# Autodesk Inventor assembly: SE Matriz Centelladora DC
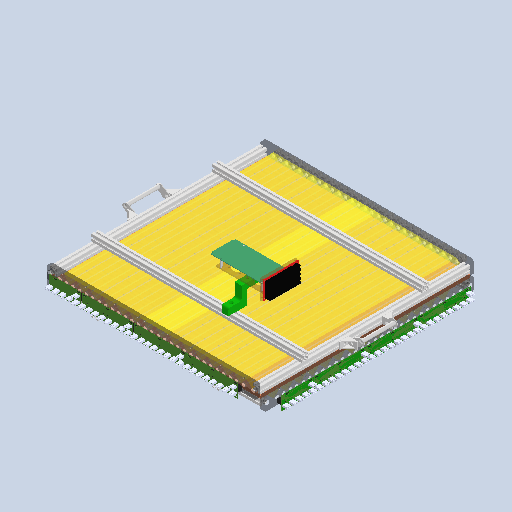
[picture p0: Inventor's stored thumbnail of the model, 512x512]
Saved by Autodesk Inventor 2024.2 (Build 282272000, 272)
## iProperties
Created: 2025-11-07
Part Number: SE Matriz Centelladora DC
Document SubType Name: Assembly
Designer: ja.restrepo1
Author: ja.restrepo1
## Documents named in this file (8)
- I:\MICROMECANICA\ALTAS ENERGIAS\Deteccion de Muones\Detectores centelladores\Partes Detector Centellador\SE Matriz Centelladora DC\SE Matriz Centelladora DC.iam
- I:\MICROMECANICA\ALTAS ENERGIAS\Deteccion de Muones\Detectores centelladores\Partes Detector Centellador\SE Matriz Centelladora DC\Soporte de matriz centelladora.ipt
- I:\MICROMECANICA\ALTAS ENERGIAS\Deteccion de Muones\Detectores centelladores\Partes Detector Centellador\SE Matriz Centelladora DC\SSE Matriz Centelladora 15X14\SSE Matriz centelladora 15X14.iam
- I:\MICROMECANICA\ALTAS ENERGIAS\Deteccion de Muones\Detectores centelladores\Partes Detector Centellador\SE Matriz Centelladora DC\SSE Estructura Centelladoras 20x20 DC\SSE estructura matriz centelladora.iam
- I:\MICROMECANICA\ALTAS ENERGIAS\Deteccion de Muones\Detectores centelladores\Partes Detector Centellador\SE Matriz Centelladora DC\SSE Manija\SSE. Manija.iam
- I:\MICROMECANICA\ALTAS ENERGIAS\Deteccion de Muones\Detectores centelladores\Partes Detector Centellador\SE Tarjetas IC DC\SSE tarjedas de AD DC.iam
- I:\MICROMECANICA\ALTAS ENERGIAS\Deteccion de Muones\Detectores centelladores\Partes Detector Centellador\SE Tarjetas IC DC\SSE SiPM 8CH Org.iam
- I:\MICROMECANICA\ALTAS ENERGIAS\Deteccion de Muones\Detectores centelladores\Partes Detector Centellador\SE Tarjetas IC DC\SSE SiPM 8Ch_2026.iam
## Components (10 placed, 7 different names)
1. Soporte de matriz centelladora:1 — Nivelación:1, Nivelación:2, Nivelación:3, Coincidencia:1, Coincidencia:2, Nivelación:4, Nivelación:5, Coincidencia:3, Nivelación:6, Nivelación:7, Coincidencia:4, Nivelación:8, Nivelación:9, Nivelación:10, Nivelación:11
2. SSE Matriz centelladora 15X14:1 [sub-assembly] — Coincidencia:2, Nivelación:4, Nivelación:6, Nivelación:7
3. SSE Matriz centelladora 15X14:2 [sub-assembly] — Nivelación:5, Coincidencia:3, Coincidencia:4
4. SSE estructura matriz centelladora:1 [sub-assembly] — Nivelación:8, Nivelación:9, Nivelación:10, Coincidencia:5, Nivelación:12, Coincidencia:6, Nivelación:13, Coincidencia:7, Ángulo:1, Nivelación:15, Coincidencia:8, Ángulo:2, Coincidencia:9, Nivelación:16, Coincidencia:10, Coincidencia:11, Nivelación:17, Nivelación:18, Coincidencia:12, Coincidencia:13
5. SSE. Manija:1 [sub-assembly] — Coincidencia:5, Nivelación:11, Nivelación:12, Nivelación:14
6. SSE. Manija:2 [sub-assembly] — Coincidencia:6, Nivelación:13, Nivelación:14
7. SSE tarjedas de AD DC:1 [sub-assembly] — Coincidencia:7, Ángulo:1, Nivelación:15
8. SSE SiPM 8CH Org:1 [sub-assembly] — Coincidencia:10, Coincidencia:11, Nivelación:17
9. SSE SiPM 8CH Org:2 [sub-assembly] — Coincidencia:8, Ángulo:2, Coincidencia:9, Nivelación:16
10. SSE SiPM 8Ch_2026:1 [sub-assembly] — Nivelación:18, Coincidencia:12, Coincidencia:13
## Relationships (33: Flush 18, Mate 13, Angle 2)
- Nivelación:1 [Flush]: Soporte de matriz centelladora:1
- Nivelación:2 [Flush]: Soporte de matriz centelladora:1
- Nivelación:3 [Flush]: Soporte de matriz centelladora:1
- Coincidencia:1 [Mate]: Soporte de matriz centelladora:1
- Coincidencia:2 [Mate]: Soporte de matriz centelladora:1 ↔ SSE Matriz centelladora 15X14:1
- Nivelación:4 [Flush]: Soporte de matriz centelladora:1 ↔ SSE Matriz centelladora 15X14:1
- Nivelación:5 [Flush]: Soporte de matriz centelladora:1 ↔ SSE Matriz centelladora 15X14:2
- Coincidencia:3 [Mate]: Soporte de matriz centelladora:1 ↔ SSE Matriz centelladora 15X14:2
- Nivelación:6 [Flush]: Soporte de matriz centelladora:1 ↔ SSE Matriz centelladora 15X14:1
- Nivelación:7 [Flush]: Soporte de matriz centelladora:1 ↔ SSE Matriz centelladora 15X14:1
- Coincidencia:4 [Mate]: Soporte de matriz centelladora:1 ↔ SSE Matriz centelladora 15X14:2
- Nivelación:8 [Flush]: Soporte de matriz centelladora:1 ↔ SSE estructura matriz centelladora:1
- Nivelación:9 [Flush]: Soporte de matriz centelladora:1 ↔ SSE estructura matriz centelladora:1
- Nivelación:10 [Flush]: Soporte de matriz centelladora:1 ↔ SSE estructura matriz centelladora:1
- Coincidencia:5 [Mate]: SSE estructura matriz centelladora:1 ↔ SSE. Manija:1
- Nivelación:11 [Flush]: Soporte de matriz centelladora:1 ↔ SSE. Manija:1
- Nivelación:12 [Flush] (0.5 mm): SSE estructura matriz centelladora:1 ↔ SSE. Manija:1
- Coincidencia:6 [Mate]: SSE estructura matriz centelladora:1 ↔ SSE. Manija:2
- Nivelación:13 [Flush] (-0.5 mm): SSE estructura matriz centelladora:1 ↔ SSE. Manija:2
- Nivelación:14 [Flush]: SSE. Manija:1 ↔ SSE. Manija:2
- Coincidencia:7 [Mate]: SSE estructura matriz centelladora:1 ↔ SSE tarjedas de AD DC:1
- Ángulo:1 [Angle] (0 deg): SSE estructura matriz centelladora:1 ↔ SSE tarjedas de AD DC:1
- Nivelación:15 [Flush] (-9 mm): SSE estructura matriz centelladora:1 ↔ SSE tarjedas de AD DC:1
- Coincidencia:8 [Mate] (10 mm): SSE estructura matriz centelladora:1 ↔ SSE SiPM 8CH Org:2
- Ángulo:2 [Angle] (0 deg): SSE estructura matriz centelladora:1 ↔ SSE SiPM 8CH Org:2
- Coincidencia:9 [Mate] (3 mm): SSE estructura matriz centelladora:1 ↔ SSE SiPM 8CH Org:2
- Nivelación:16 [Flush]: SSE estructura matriz centelladora:1 ↔ SSE SiPM 8CH Org:2
- Coincidencia:10 [Mate] (10 mm): SSE estructura matriz centelladora:1 ↔ SSE SiPM 8CH Org:1
- Coincidencia:11 [Mate] (3 mm): SSE estructura matriz centelladora:1 ↔ SSE SiPM 8CH Org:1
- Nivelación:17 [Flush]: SSE estructura matriz centelladora:1 ↔ SSE SiPM 8CH Org:1
- Nivelación:18 [Flush]: SSE estructura matriz centelladora:1 ↔ SSE SiPM 8Ch_2026:1
- Coincidencia:12 [Mate] (10 mm): SSE estructura matriz centelladora:1 ↔ SSE SiPM 8Ch_2026:1
- Coincidencia:13 [Mate]: SSE estructura matriz centelladora:1 ↔ SSE SiPM 8Ch_2026:1
